# Autodesk Inventor assembly: DFPlayer Mini
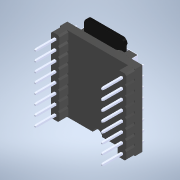
[picture p0: Inventor's stored thumbnail of the model, 180x180]
Saved by Autodesk Inventor 2021 (Build 250183000, 183)
## iProperties
Created: 2023-08-06
Part Number: DFPlayer Mini
Document SubType Name: Assembly
Designer: michal
Author: michal
## Documents named in this file (3)
- C:\Users\micha\OneDrive\Dokumenty\GitHub\escape_room_hw_v2\Enclosure\Commercial\DFPlayer Mini.iam
- C:\Users\micha\OneDrive\Dokumenty\GitHub\escape_room_hw_v2\Enclosure\Commercial\DFR0299.ipt
- C:\Users\micha\OneDrive\Dokumenty\GitHub\escape_room_hw_v2\Enclosure\Commercial\Micro SD Card.ipt
## Components (2 placed, 2 different names)
1. DFR0299:1 — Mate:1, Mate:2, Flush:1
2. Micro SD Card:1 — Mate:1, Mate:2, Flush:1
## Relationships (3: Mate 2, Flush 1)
- Mate:1: DFR0299:1 ↔ Micro SD Card:1
- Mate:2: DFR0299:1 ↔ Micro SD Card:1
- Flush:1 (-2.5 mm): DFR0299:1 ↔ Micro SD Card:1
